# Autodesk Inventor assembly: magnets
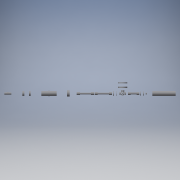
[picture p0: Inventor's stored thumbnail of the model, 180x180]
Saved by Autodesk Inventor 2019 (Build 230136000, 136)
## iProperties
Created: 2019-07-25
Part Number: magnets
Document SubType Name: Assembly
Designer: afelepar
Author: afelepar
## Documents named in this file (44)
- C:\Ali Fele paranj\Magnets_Original\magnets.iam
- C:\Ali Fele paranj\Magnets_Original\AGBL07-1.ipt
- C:\Ali Fele paranj\Magnets_Original\AGBL07-2.ipt
- C:\Ali Fele paranj\Magnets_Original\AGBL06.ipt
- C:\Ali Fele paranj\Magnets_Original\AGBL06_2.ipt
- C:\Ali Fele paranj\Magnets_Original\AGBL01-1.ipt
- C:\Ali Fele paranj\Magnets_Original\AGBL01-1_2.ipt
- C:\Ali Fele paranj\Magnets_Original\AGBL02.ipt
- C:\Ali Fele paranj\Magnets_Original\AGBL02_2.ipt
- C:\Ali Fele paranj\Magnets_Original\AGBL02_3.ipt
- C:\Ali Fele paranj\Magnets_Original\AGBL02_4.ipt
- C:\Ali Fele paranj\Magnets_Original\AGBL02_5.ipt
- C:\Ali Fele paranj\Magnets_Original\ALPHA-II-CT.ipt
- C:\Ali Fele paranj\Magnets_Original\ALPHA-II-CT_2.ipt
- C:\Ali Fele paranj\Magnets_Original\ALPHA-II-CT_3.ipt
- C:\Ali Fele paranj\Magnets_Original\ALPHA-II-CT_4.ipt
- C:\Ali Fele paranj\Magnets_Original\ALPHA-II-CT_5.ipt
- C:\Ali Fele paranj\Magnets_Original\ALPHA-II-CT_6.ipt
- C:\Ali Fele paranj\Magnets_Original\ALPHA-II-CT_7.ipt
- C:\Ali Fele paranj\Magnets_Original\ALPHA-II-CT_8.ipt
- C:\Ali Fele paranj\Magnets_Original\ALPHA-II-CT_9.ipt
- C:\Ali Fele paranj\Magnets_Original\ALPHA-II-CT_10.ipt
- C:\Ali Fele paranj\Magnets_Original\ALPHA-II-CT_11.ipt
- C:\Ali Fele paranj\Magnets_Original\ALPHA-II-CT_12.ipt
- C:\Ali Fele paranj\Magnets_Original\ALPHA-II-T2.ipt
- C:\Ali Fele paranj\Magnets_Original\ALPHA-II-T3.ipt
- C:\Ali Fele paranj\Magnets_Original\ALPHA-II-T4.ipt
- C:\Ali Fele paranj\Magnets_Original\ALPHA-II-AT.ipt
- C:\Ali Fele paranj\Magnets_Original\ALPHA-II-AT_2.ipt
- C:\Ali Fele paranj\Magnets_Original\ALPHA-II-AT_3.ipt
- C:\Ali Fele paranj\Magnets_Original\ALPHA-II-AT_4.ipt
- C:\Ali Fele paranj\Magnets_Original\ALPHA-II-AT_5.ipt
- C:\Ali Fele paranj\Magnets_Original\AGBL03.ipt
- C:\Ali Fele paranj\Magnets_Original\AGBL03_2.ipt
- C:\Ali Fele paranj\Magnets_Original\AGBL08.ipt
- C:\Ali Fele paranj\Magnets_Original\AGBL08_2.ipt
- C:\Ali Fele paranj\Magnets_Original\AGBL04.ipt
- C:\Ali Fele paranj\Magnets_Original\AGBL04_2.ipt
- C:\Ali Fele paranj\Magnets_Original\AGBL05.ipt
- C:\Ali Fele paranj\Magnets_Original\POSITRONS.ipt
- C:\Ali Fele paranj\Magnets_Original\AGBL03_REV_01.ipt
- C:\Ali Fele paranj\Magnets_Original\AGBL03_REV_01_2.ipt
- C:\Ali Fele paranj\Magnets_Original\AGBL01_2_REV_00.ipt
- C:\Ali Fele paranj\Magnets_Original\PULSED_TRANSFER.ipt
## Components (44 placed, 44 different names)
1. AGBL07-1:1 — Mate:2, Angle:2
2. AGBL07-2:1 — Mate:1, Angle:1
3. AGBL06:1 — Mate:3, Mate:4
4. AGBL06_2:1 — Mate:5, Mate:6
5. AGBL01-1:1 — Mate:7, Mate:8
6. AGBL01-1_2:1 — Mate:9, Mate:10
7. AGBL02:1 — Mate:11, Mate:12
8. AGBL02_2:1 — Mate:13, Mate:14
9. AGBL02_3:1 — Mate:15, Mate:16
10. AGBL02_4:1 — Mate:17, Mate:18
11. AGBL02_5:1 — Mate:19, Mate:20
12. AGBL02_6:2 — Mate:21, Mate:22
13. ALPHA-II-CT:1 — Mate:23, Mate:24
14. ALPHA-II-CT_2:1 — Mate:25, Mate:26
15. ALPHA-II-CT_3:1 — Mate:27, Mate:28
16. ALPHA-II-CT_4:1 — Mate:29, Mate:30
17. ALPHA-II-CT_5:1
18. ALPHA-II-CT_6:1 — Mate:33, Mate:34
19. ALPHA-II-CT_7:1 — Mate:35, Mate:36
20. ALPHA-II-CT_8:1 — Mate:37, Mate:38
21. ALPHA-II-CT_9:1 — Mate:39, Mate:40
22. ALPHA-II-CT_10:1 — Mate:41, Mate:42
23. ALPHA-II-CT_11:1 — Mate:43, Mate:44
24. ALPHA-II-CT_12:1 — Mate:45, Mate:46
25. ALPHA-II-T2:1 — Mate:47, Mate:48
26. ALPHA-II-T3:1 — Mate:49, Mate:50
27. ALPHA-II-T4:1 — Mate:51, Mate:52
28. ALPHA-II-AT:1 — Mate:53, Mate:54
29. ALPHA-II-AT_2:1 — Mate:55, Mate:56
30. ALPHA-II-AT_3:1 — Mate:57, Mate:58
31. ALPHA-II-AT_4:1 — Mate:59, Mate:60
32. ALPHA-II-AT_5:1 — Mate:61, Mate:62
33. AGBL03:1 — Mate:63, Mate:67
34. AGBL03_2:1 — Mate:65, Mate:68
35. AGBL08:1 — Mate:69, Mate:70
36. AGBL08_2:1 — Mate:71, Mate:72
37. AGBL04:1 — Mate:73, Mate:74
38. AGBL04_2:1 — Mate:75, Mate:76
39. AGBL05:1 — Mate:78, Mate:79
40. POSITRONS:1 — Mate:80, Mate:81
41. AGBL03_REV_01:1 — Mate:82, Mate:83
42. AGBL03_REV_01_2:1 — Mate:84, Mate:85
43. AGBL01_2_REV_00:1 — Mate:86, Mate:87
44. PULSED_TRANSFER:1 — Mate:88, Mate:89
## Relationships (86: Mate 84, Angle 2)
- Mate:1: AGBL07-2:1
- Angle:1 (-45 deg): AGBL07-2:1
- Mate:2: AGBL07-1:1
- Angle:2 (-45 deg): AGBL07-1:1
- Mate:3: AGBL06:1
- Mate:4 (210 mm): AGBL06:1
- Mate:5 (210 mm): AGBL06_2:1
- Mate:6: AGBL06_2:1
- Mate:7 (1425.5 mm): AGBL01-1:1
- Mate:8: AGBL01-1:1
- Mate:9 (2812.7 mm): AGBL01-1_2:1
- Mate:10: AGBL01-1_2:1
- Mate:11 (3426.519 mm): AGBL02:1
- Mate:12: AGBL02:1
- Mate:13 (2323.881 mm): AGBL02_2:1
- Mate:14: AGBL02_2:1
- Mate:15 (2039.319 mm): AGBL02_3:1
- Mate:16: AGBL02_3:1
- Mate:17 (936.681 mm): AGBL02_4:1
- Mate:18: AGBL02_4:1
- Mate:19 (509.263 mm): AGBL02_5:1
- Mate:20: AGBL02_5:1
- Mate:21 (1187.237 mm): AGBL02_6:2
- Mate:22: AGBL02_6:2
- Mate:23 (-8856.9 mm): ALPHA-II-CT:1
- Mate:24: ALPHA-II-CT:1
- Mate:25 (-8856.9 mm): ALPHA-II-CT_2:1
- Mate:26: ALPHA-II-CT_2:1
- Mate:27 (-8856.9 mm): ALPHA-II-CT_3:1
- Mate:28: ALPHA-II-CT_3:1
- Mate:29 (-8856.9 mm): ALPHA-II-CT_4:1
- Mate:30: ALPHA-II-CT_4:1
- Mate:33 (-8856.9 mm): ALPHA-II-CT_6:1
- Mate:34: ALPHA-II-CT_6:1
- Mate:35 (-8856.9 mm): ALPHA-II-CT_7:1
- Mate:36: ALPHA-II-CT_7:1
- Mate:37 (-8856.9 mm): ALPHA-II-CT_8:1
- Mate:38: ALPHA-II-CT_8:1
- Mate:39 (-8856.9 mm): ALPHA-II-CT_9:1
- Mate:40: ALPHA-II-CT_9:1
- Mate:41 (-8856.9 mm): ALPHA-II-CT_10:1
- Mate:42: ALPHA-II-CT_10:1
- Mate:43 (-8856.9 mm): ALPHA-II-CT_11:1
- Mate:44: ALPHA-II-CT_11:1
- Mate:45 (-8856.9 mm): ALPHA-II-CT_12:1
- Mate:46: ALPHA-II-CT_12:1
- Mate:47 (-7658.6 mm): ALPHA-II-T2:1
- Mate:48: ALPHA-II-T2:1
- Mate:49 (-7155.6 mm): ALPHA-II-T3:1
- Mate:50: ALPHA-II-T3:1
- Mate:51 (4187 mm): ALPHA-II-T4:1
- Mate:52: ALPHA-II-T4:1
- Mate:53 (-5679.9 mm): ALPHA-II-AT:1
- Mate:54: ALPHA-II-AT:1
- Mate:55 (-5679.9 mm): ALPHA-II-AT_2:1
- Mate:56: ALPHA-II-AT_2:1
- Mate:57 (-5679.9 mm): ALPHA-II-AT_3:1
- Mate:58: ALPHA-II-AT_3:1
- Mate:59 (5679.9 mm): ALPHA-II-AT_4:1
- Mate:60: ALPHA-II-AT_4:1
- Mate:61 (-5679.9 mm): ALPHA-II-AT_5:1
- Mate:62: ALPHA-II-AT_5:1
- Mate:63 (-715 mm): AGBL03:1
- Mate:65 (-455 mm): AGBL03_2:1
- Mate:67: AGBL03:1
- Mate:68: AGBL03_2:1
- Mate:69 (820 mm): AGBL08:1
- Mate:70: AGBL08:1
- Mate:71 (475 mm): AGBL08_2:1
- Mate:72: AGBL08_2:1
- Mate:73 (-202.5 mm): AGBL04:1
- Mate:74: AGBL04:1
- Mate:75 (202.5 mm): AGBL04_2:1
- Mate:76: AGBL04_2:1
- Mate:78: AGBL05:1
- Mate:79 (194.5 mm): AGBL05:1
- Mate:80 (3187.83 mm): POSITRONS:1
- Mate:81: POSITRONS:1
- Mate:82 (1622.807 mm): AGBL03_REV_01:1
- Mate:83: AGBL03_REV_01:1
- Mate:84 (1362.807 mm): AGBL03_REV_01_2:1
- Mate:85: AGBL03_REV_01_2:1
- Mate:86 (848.25 mm): AGBL01_2_REV_00:1
- Mate:87: AGBL01_2_REV_00:1
- Mate:88 (1829 mm): PULSED_TRANSFER:1
- Mate:89: PULSED_TRANSFER:1
